# Autodesk Inventor assembly: цепь
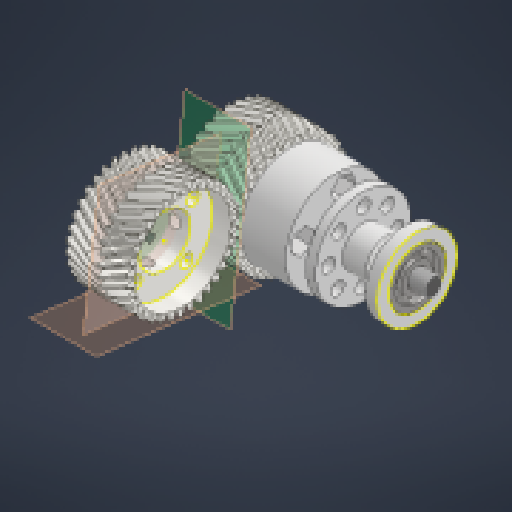
[picture p0: Inventor's stored thumbnail of the model, 512x512]
Saved by Autodesk Inventor 2025 (Build 290162000, 162)
## iProperties
Created: 2024-07-09
Part Number: цепь
Document SubType Name: Assembly
Designer: Phantom
Author: Phantom
## Documents named in this file (6)
- C:\Users\Phantom\Desktop\Phantom16950\цепь.iam
- C:\Users\Phantom\Desktop\Phantom16950\втулка для подш 2 часть.ipt
- C:\Users\Phantom\Desktop\Phantom16950\втулка для подш.ipt
- C:\Users\Phantom\Desktop\Phantom16950\Деталь_64.ipt
- C:\Users\Phantom\Desktop\Phantom16950\BS 290 SKF - SKF 626-RZ.ipt
- C:\Users\Phantom\Desktop\Phantom16950\цепь\Мастер проектирования\Цилиндрическое зубчатое зацепление4.iam
## Components (6 placed, 5 different names)
1. втулка для подш 2 часть:1 — Совмещение:16, Совмещение:20, Совмещение:23
2. втулка для подш:1 — Совмещение:16, Совмещение:17, Совмещение:25, Совмещение:26
3. Деталь_64:1 — Совмещение:17, Совмещение:19, Совмещение:21, Совмещение:23
4. BS 290 SKF - SKF 626-RZ:1 — Совмещение:20, Совмещение:21
5. BS 290 SKF - SKF 626-RZ:2 — Совмещение:19, Совмещение:27
6. Цилиндрическое зубчатое зацепление:4 [sub-assembly] — Совмещение:25, Совмещение:26, Совмещение:27
## Relationships (9: Mate 9)
- Совмещение:16 [Mate]: втулка для подш 2 часть:1 ↔ втулка для подш:1
- Совмещение:17 [Mate]: втулка для подш:1 ↔ Деталь_64:1
- Совмещение:19 [Mate]: Деталь_64:1 ↔ BS 290 SKF - SKF 626-RZ:2
- Совмещение:20 [Mate]: втулка для подш 2 часть:1 ↔ BS 290 SKF - SKF 626-RZ:1
- Совмещение:21 [Mate]: Деталь_64:1 ↔ BS 290 SKF - SKF 626-RZ:1
- Совмещение:23 [Mate]: втулка для подш 2 часть:1 ↔ Деталь_64:1
- Совмещение:25 [Mate]: втулка для подш:1 ↔ Цилиндрическое зубчатое зацепление:4
- Совмещение:26 [Mate]: втулка для подш:1 ↔ Цилиндрическое зубчатое зацепление:4
- Совмещение:27 [Mate]: BS 290 SKF - SKF 626-RZ:2 ↔ Цилиндрическое зубчатое зацепление:4
